# Autodesk Inventor assembly: единое крепление
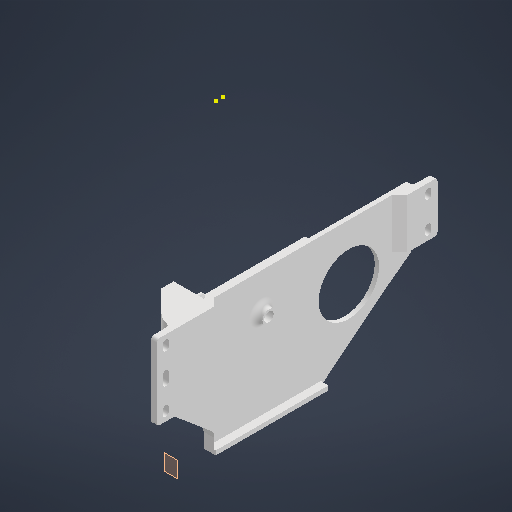
[picture p0: Inventor's stored thumbnail of the model, 512x512]
Saved by Autodesk Inventor 2025 (Build 290162000, 162)
## iProperties
Created: 2024-09-25
Part Number: единое крепление
Document SubType Name: Assembly
Designer: GameHD
Author: GameHD
## Documents named in this file (3)
- C:\Users\Phantom\Desktop\Phantom16950\единое крепление.iam
- C:\Users\Phantom\Desktop\Phantom16950\крепл для колёс.ipt
- C:\Users\Phantom\Desktop\Phantom16950\крепл для колёс. 2 часть.ipt
## Components (2 placed, 2 different names)
1. крепл для колёс:1 — Совмещение:4, Заподлицо:5
2. крепл для колёс. 2 часть:1 — Совмещение:4, Заподлицо:5
## Relationships (2: Mate 1, Flush 1)
- Совмещение:4 [Mate]: крепл для колёс:1 ↔ крепл для колёс. 2 часть:1
- Заподлицо:5 [Flush]: крепл для колёс:1 ↔ крепл для колёс. 2 часть:1
